# Autodesk Inventor assembly: hinge asembaly (new)
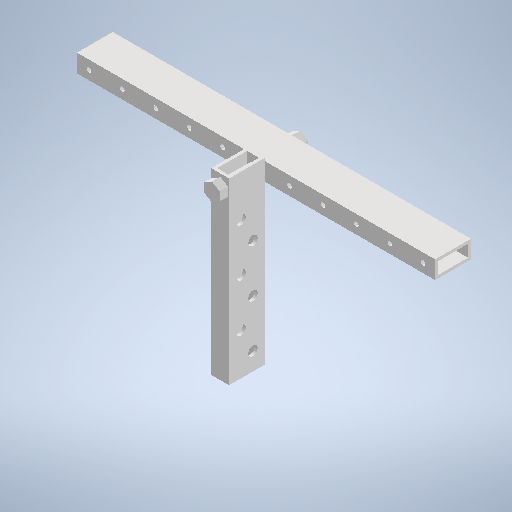
[picture p0: Inventor's stored thumbnail of the model, 512x512]
Saved by Autodesk Inventor 2025.2 (Build 292293000, 293)
## iProperties
Created: 2025-01-08
Part Number: hinge asembaly (new)
Document SubType Name: Assembly
Designer: 5013908
Author: 5013908
## Documents named in this file (4)
- C:\Users\5013908\Documents\GitHub\Mechanical\SeattleSolarCar2024-2025\Frame\hinge asembaly (new).iam
- C:\Users\5013908\Documents\GitHub\Mechanical\SeattleSolarCar2024-2025\Frame\hinge base.ipt
- C:\Users\5013908\Documents\GitHub\Mechanical\SeattleSolarCar2024-2025\Frame\hing rod.ipt
- C:\Users\5013908\Documents\GitHub\Mechanical\SeattleSolarCar2024-2025\Frame\hinge aray side.ipt
## Components (3 placed, 3 different names)
1. hinge base:1 — Rotational:1
2. hing rod:1 — Rotational:1, Rotational:2
3. hinge aray side:1 — Rotational:2
## Relationships (2: RevoluteJoint 2)
- Rotational:1 [RevoluteJoint]: hinge base:1 ↔ hing rod:1
- Rotational:2 [RevoluteJoint]: hing rod:1 ↔ hinge aray side:1
